# Autodesk Inventor assembly: dash-
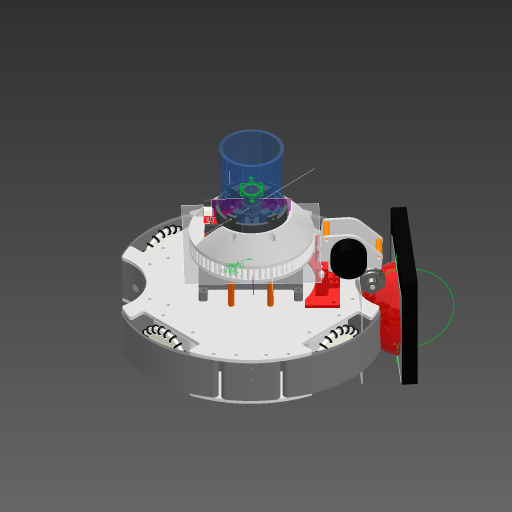
[picture p0: Inventor's stored thumbnail of the model, 512x512]
Saved by Autodesk Inventor 2023 (Build 270158000, 158)
## iProperties
Created: 2025-06-27
Part Number: dash-
Document SubType Name: Assembly
Designer: daa
Author: daa
## Documents named in this file (10)
- C:\Users\daa\Documents\DASH_V2\dash-.iam
- C:\Users\daa\Documents\DASH_V2\omni_platforma\omni_platforma.iam
- C:\Users\daa\Documents\DASH_V2\omni_platforma\top.ipt
- C:\Users\daa\Documents\DASH_V2\omni_platforma\akb.ipt
- C:\Users\daa\Documents\DASH_V2\Stoics.ipt
- C:\Users\daa\Documents\DASH_V2\tower.iam
- C:\Users\daa\Documents\DASH_V2\Dribler_v2\kreplenie_dribler_V3.ipt
- C:\Users\daa\Documents\DASH_V2\Dribler_v2\axis.ipt
- C:\Users\daa\Documents\DASH_V2\dribler.iam
- C:\Users\daa\Documents\DASH_V2\ball_2.ipt
## Components (12 placed, 9 different names)
1. omni_platforma:1 [sub-assembly] — С поворотом:1
2. top:1 — С поворотом:1, С поворотом:2, Жесткий:1, Жесткий:2, Жесткий:3, Жесткий:4, С поворотом:4
3. akb:2 — С поворотом:2
4. Stoics:1 — Жесткий:2
5. Stoics:2 — Жесткий:1, С поворотом:3
6. Stoics:3 — Жесткий:3
7. Stoics:4 — Жесткий:4
8. tower:1 [sub-assembly] — С поворотом:3
9. kreplenie_dribler_V3:1 — С поворотом:4, С поворотом:5
10. axis:1 — С поворотом:5, Вставка:1
11. dribler:1 [sub-assembly] — Вставка:1
12. ball_2:1
## Relationships (10: RevoluteJoint 5, WeldJoint 4, Insert 1)
- С поворотом:1 [RevoluteJoint]: omni_platforma:1 ↔ top:1
- С поворотом:2 [RevoluteJoint]: top:1 ↔ akb:2
- Жесткий:1 [WeldJoint]: top:1 ↔ Stoics:2
- Жесткий:2 [WeldJoint]: top:1 ↔ Stoics:1
- Жесткий:3 [WeldJoint]: top:1 ↔ Stoics:3
- Жесткий:4 [WeldJoint]: top:1 ↔ Stoics:4
- С поворотом:3 [RevoluteJoint]: Stoics:2 ↔ tower:1
- С поворотом:4 [RevoluteJoint]: top:1 ↔ kreplenie_dribler_V3:1
- С поворотом:5 [RevoluteJoint] (-15 mm): kreplenie_dribler_V3:1 ↔ axis:1
- Вставка:1 [Insert] (-17.5 mm): axis:1 ↔ dribler:1
